# Autodesk Inventor assembly: ASY NVPH-400 shredder
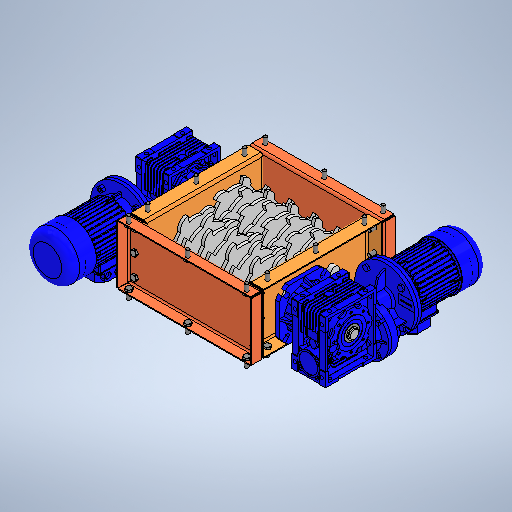
[picture p0: Inventor's stored thumbnail of the model, 512x512]
Saved by Autodesk Inventor 2025.1 (Build 291241020, 241B)
## iProperties
Created: 2024-12-13
Part Number: ASY NVPH-400 shredder
Document SubType Name: Assembly
Designer: user
Author: user
## Documents named in this file (6)
- C:\Users\user\YandexDisk-badmisterfox\домашниий пк\Inventor\NDM-VOS_powder_hopper\ASY NVPH-400 shredder.iam
- C:\Users\user\YandexDisk-badmisterfox\домашниий пк\Inventor\NDM-VOS_powder_hopper\ASY NVPH-200 shredder shaft full.iam
- C:\Users\user\YandexDisk-badmisterfox\домашниий пк\Inventor\NDM-VOS_powder_hopper\NDM-VOS 111 sredder wall .ipt
- C:\Users\user\YandexDisk-badmisterfox\домашниий пк\Inventor\NDM-VOS_powder_hopper\3d party\PCRV080-075SHFA_MS80B5\PCRV080-075SHFA_MS80B5\PCRV080-075SHFA_MS80B5.ipt
- C:\Users\user\YandexDisk-badmisterfox\домашниий пк\Inventor\NDM-VOS_powder_hopper\NDM-VOS 111 sredder wall _CPY.ipt
- C:\Users\user\YandexDisk-badmisterfox\домашниий пк\Inventor\Content Center Files\en-US\ISO 4017(1)\ISO 4017 - M12 x 25 - ISO.ipt
## Components (44 placed, 5 different names)
1. ASY NVPH-200 shredder shaft full:1 [sub-assembly] — Rotational:1
2. ASY NVPH-200 shredder shaft full:2 [sub-assembly] — Rotational:2
3. NDM-VOS 111 sredder wall :1 — Rigid:1, Rigid:3, Insert:13, Insert:14, Insert:15, Insert:16, Insert:17, Insert:18, Flush:1, Rotational:1, Rigid:4
4. NDM-VOS 111 sredder wall :2 — Rigid:2, Insert:19, Insert:20, Insert:21, Insert:22, Insert:23, Insert:24, Rotational:2, Rigid:5
5. PCRV080-075SHFA_MS80B5:1 — Rigid:4
6. PCRV080-075SHFA_MS80B5:2 — Rigid:5
7. NDM-VOS 112 sredder wall sub:1 — Rigid:1, Rigid:2, Insert:1, Insert:2, Insert:3, Insert:4, Insert:5, Insert:6, Insert:7, Insert:8, Insert:9, Insert:10, Insert:11, Insert:12, Mate:1, Mate:2
8. NDM-VOS 112 sredder wall sub:2 — Rigid:3, Insert:25, Insert:26, Insert:27, Insert:28, Insert:29, Insert:30, Insert:31, Insert:32, Insert:33, Insert:34, Insert:35, Insert:36
9. ISO 4017 M12 x 25:1 — Insert:1
10. ISO 4017 M12 x 25:2 — Insert:2
11. ISO 4017 M12 x 25:3 — Insert:3
12. ISO 4017 M12 x 25:4 — Insert:4
13. ISO 4017 M12 x 25:5 — Insert:5
14. ISO 4017 M12 x 25:6 — Insert:6
15. ISO 4017 M12 x 25:7 — Insert:7
16. ISO 4017 M12 x 25:8 — Insert:8
17. ISO 4017 M12 x 25:9 — Insert:9
18. ISO 4017 M12 x 25:10 — Insert:10
19. ISO 4017 M12 x 25:11 — Insert:11
20. ISO 4017 M12 x 25:12 — Insert:12
21. ISO 4017 M12 x 25:13 — Insert:13
22. ISO 4017 M12 x 25:14 — Insert:14
23. ISO 4017 M12 x 25:15 — Insert:15
24. ISO 4017 M12 x 25:16 — Insert:16
25. ISO 4017 M12 x 25:17 — Insert:17
26. ISO 4017 M12 x 25:18 — Insert:18
27. ISO 4017 M12 x 25:19 — Insert:19
28. ISO 4017 M12 x 25:20 — Insert:20
29. ISO 4017 M12 x 25:21 — Insert:21
30. ISO 4017 M12 x 25:22 — Insert:22
31. ISO 4017 M12 x 25:23 — Insert:23
32. ISO 4017 M12 x 25:24 — Insert:24
33. ISO 4017 M12 x 25:25 — Insert:25
34. ISO 4017 M12 x 25:26 — Insert:26
35. ISO 4017 M12 x 25:27 — Insert:27
36. ISO 4017 M12 x 25:28 — Insert:28
37. ISO 4017 M12 x 25:29 — Insert:29
38. ISO 4017 M12 x 25:30 — Insert:30
39. ISO 4017 M12 x 25:31 — Insert:31
40. ISO 4017 M12 x 25:32 — Insert:32
41. ISO 4017 M12 x 25:33 — Insert:33
42. ISO 4017 M12 x 25:34 — Insert:34
43. ISO 4017 M12 x 25:35 — Insert:35
44. ISO 4017 M12 x 25:36 — Insert:36
## Relationships (46: Insert 36, WeldJoint 5, Mate 2, RevoluteJoint 2, Flush 1)
- Rigid:1 [WeldJoint]: NDM-VOS 111 sredder wall :1 ↔ NDM-VOS 112 sredder wall sub:1
- Rigid:2 [WeldJoint]: NDM-VOS 111 sredder wall :2 ↔ NDM-VOS 112 sredder wall sub:1
- Rigid:3 [WeldJoint]: NDM-VOS 111 sredder wall :1 ↔ NDM-VOS 112 sredder wall sub:2
- Insert:1: NDM-VOS 112 sredder wall sub:1 ↔ ISO 4017 M12 x 25:1
- Insert:2: NDM-VOS 112 sredder wall sub:1 ↔ ISO 4017 M12 x 25:2
- Insert:3: NDM-VOS 112 sredder wall sub:1 ↔ ISO 4017 M12 x 25:3
- Insert:4: NDM-VOS 112 sredder wall sub:1 ↔ ISO 4017 M12 x 25:4
- Insert:5: NDM-VOS 112 sredder wall sub:1 ↔ ISO 4017 M12 x 25:5
- Insert:6: NDM-VOS 112 sredder wall sub:1 ↔ ISO 4017 M12 x 25:6
- Insert:7: NDM-VOS 112 sredder wall sub:1 ↔ ISO 4017 M12 x 25:7
- Insert:8: NDM-VOS 112 sredder wall sub:1 ↔ ISO 4017 M12 x 25:8
- Insert:9: NDM-VOS 112 sredder wall sub:1 ↔ ISO 4017 M12 x 25:9
- Insert:10: NDM-VOS 112 sredder wall sub:1 ↔ ISO 4017 M12 x 25:10
- Insert:11: NDM-VOS 112 sredder wall sub:1 ↔ ISO 4017 M12 x 25:11
- Insert:12: NDM-VOS 112 sredder wall sub:1 ↔ ISO 4017 M12 x 25:12
- Insert:13: NDM-VOS 111 sredder wall :1 ↔ ISO 4017 M12 x 25:13
- Insert:14: NDM-VOS 111 sredder wall :1 ↔ ISO 4017 M12 x 25:14
- Insert:15: NDM-VOS 111 sredder wall :1 ↔ ISO 4017 M12 x 25:15
- Insert:16: NDM-VOS 111 sredder wall :1 ↔ ISO 4017 M12 x 25:16
- Insert:17: NDM-VOS 111 sredder wall :1 ↔ ISO 4017 M12 x 25:17
- Insert:18: NDM-VOS 111 sredder wall :1 ↔ ISO 4017 M12 x 25:18
- Insert:19: NDM-VOS 111 sredder wall :2 ↔ ISO 4017 M12 x 25:19
- Insert:20: NDM-VOS 111 sredder wall :2 ↔ ISO 4017 M12 x 25:20
- Insert:21: NDM-VOS 111 sredder wall :2 ↔ ISO 4017 M12 x 25:21
- Insert:22: NDM-VOS 111 sredder wall :2 ↔ ISO 4017 M12 x 25:22
- Insert:23: NDM-VOS 111 sredder wall :2 ↔ ISO 4017 M12 x 25:23
- Insert:24: NDM-VOS 111 sredder wall :2 ↔ ISO 4017 M12 x 25:24
- Insert:25: NDM-VOS 112 sredder wall sub:2 ↔ ISO 4017 M12 x 25:25
- Insert:26: NDM-VOS 112 sredder wall sub:2 ↔ ISO 4017 M12 x 25:26
- Insert:27: NDM-VOS 112 sredder wall sub:2 ↔ ISO 4017 M12 x 25:27
- Insert:28: NDM-VOS 112 sredder wall sub:2 ↔ ISO 4017 M12 x 25:28
- Insert:29: NDM-VOS 112 sredder wall sub:2 ↔ ISO 4017 M12 x 25:29
- Insert:30: NDM-VOS 112 sredder wall sub:2 ↔ ISO 4017 M12 x 25:30
- Insert:31: NDM-VOS 112 sredder wall sub:2 ↔ ISO 4017 M12 x 25:31
- Insert:32: NDM-VOS 112 sredder wall sub:2 ↔ ISO 4017 M12 x 25:32
- Insert:33: NDM-VOS 112 sredder wall sub:2 ↔ ISO 4017 M12 x 25:33
- Insert:34: NDM-VOS 112 sredder wall sub:2 ↔ ISO 4017 M12 x 25:34
- Insert:35: NDM-VOS 112 sredder wall sub:2 ↔ ISO 4017 M12 x 25:35
- Insert:36: NDM-VOS 112 sredder wall sub:2 ↔ ISO 4017 M12 x 25:36
- Mate:1: NDM-VOS 112 sredder wall sub:1
- Mate:2: NDM-VOS 112 sredder wall sub:1
- Flush:1: NDM-VOS 111 sredder wall :1
- Rotational:1 [RevoluteJoint] (-2 mm): ASY NVPH-200 shredder shaft full:1 ↔ NDM-VOS 111 sredder wall :1
- Rotational:2 [RevoluteJoint] (-2 mm): ASY NVPH-200 shredder shaft full:2 ↔ NDM-VOS 111 sredder wall :2
- Rigid:4 [WeldJoint] (-50 mm): NDM-VOS 111 sredder wall :1 ↔ PCRV080-075SHFA_MS80B5:1
- Rigid:5 [WeldJoint] (50 mm): NDM-VOS 111 sredder wall :2 ↔ PCRV080-075SHFA_MS80B5:2
